# Autodesk Inventor assembly: panelsWithKerf
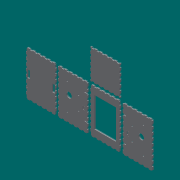
[picture p0: Inventor's stored thumbnail of the model, 180x180]
Saved by Autodesk Inventor 2016 (Build 200138000, 138)
## iProperties
Created: 2016-09-07
Part Number: panelsWithKerf
Document SubType Name: Assembly
Designer: sawaiz
Author: sawaiz
## Documents named in this file (7)
- C:\Users\sawaiz\oneDrive\projects\splitFlapDisplay\panelsWithKerf.iam
- C:\Users\sawaiz\oneDrive\projects\splitFlapDisplay\frame\front.ipt
- C:\Users\sawaiz\oneDrive\projects\splitFlapDisplay\frame\topBottomPanel.ipt
- C:\Users\sawaiz\oneDrive\projects\splitFlapDisplay\frame\leftSide.ipt
- C:\Users\sawaiz\oneDrive\projects\splitFlapDisplay\frame\rightSide.ipt
- C:\Users\sawaiz\oneDrive\projects\splitFlapDisplay\frame\back.ipt
- C:\Users\sawaiz\oneDrive\projects\splitFlapDisplay\panelsWithKerf.ipt
## Components (6 placed, 6 different names)
1. front:1 — Flush:1, Flush:2, Flush:3, Flush:4, Flush:5, Flush:6, Flush:7, Flush:9
2. topBottomPanel:1 — Flush:3, Flush:5
3. leftSide:1 — Flush:2, Flush:7, Flush:8
4. rightSide:1 — Flush:4, Flush:6
5. back:1 — Flush:1, Flush:8
6. panelsWithKerf:1 — Flush:9
## Relationships (9: Flush 9)
- Flush:1: front:1 ↔ back:1
- Flush:2: front:1 ↔ leftSide:1
- Flush:3: front:1 ↔ topBottomPanel:1
- Flush:4: front:1 ↔ rightSide:1
- Flush:5: front:1 ↔ topBottomPanel:1
- Flush:6: front:1 ↔ rightSide:1
- Flush:7: front:1 ↔ leftSide:1
- Flush:8: leftSide:1 ↔ back:1
- Flush:9: front:1 ↔ panelsWithKerf:1
